# Autodesk Inventor assembly: Assembly
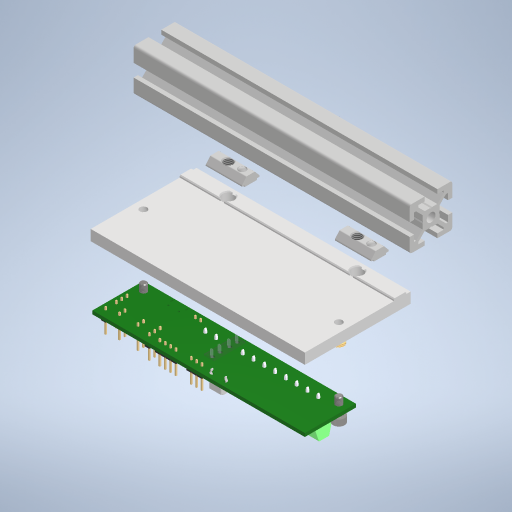
[picture p0: Inventor's stored thumbnail of the model, 512x512]
Saved by Autodesk Inventor 2023.1 (Build 271208000, 208)
## iProperties
Created: 2022-09-11
Part Number: Assembly
Document SubType Name: Assembly
Designer: Rama
Author: Rama
## Documents named in this file (8)
- C:\Users\Rama\Desktop\Mix\Klipper_Expander\CAD\Source\Assembly.iam
- C:\Users\Rama\Desktop\Mix\Klipper_Expander\CAD\Source\Klipper_Expander_Mount.ipt
- C:\Users\Rama\Documents\Inventor\Content Center Files\R2023\de-DE\ISO 7380-1\ISO 7380-1 - M5 x 8.ipt
- C:\Users\Rama\Desktop\GitHub\TrashInventor\HFSB5-2020-130.ipt
- C:\Users\Rama\Documents\Inventor\Content Center Files\R2023\de-DE\DIN 912\DIN 912 - M3 x 0,5 x 8 x 6,75.ipt
- C:\Users\Rama\Desktop\GitHub\TrashInventor\M3 Threaded Insert.ipt
- C:\Users\Rama\Desktop\GitHub\TrashInventor\SHNTP5-5.ipt
- C:\Users\Rama\Desktop\KE\STM32_Klipper_Expander.iam
## Components (11 placed, 7 different names)
1. Klipper_Expander_Mount:1 — Passend:1, Passend:2, Passend:7, Passend:8, Fluchtend:6
2. ISO 7380-1 M5 x 8:1 — Passend:1, Fluchtend:1, Passend:9
3. ISO 7380-1 M5 x 8:2 — Passend:2, Fluchtend:1, Passend:10
4. HFSB5-2020-130:1 — Passend:11, Winkel:1, Fluchtend:6
5. DIN 912 - ersetzt durch DIN EN ISO 4762 M3 x 8:1 — Fluchtend:2
6. DIN 912 - ersetzt durch DIN EN ISO 4762 M3 x 8:2 — Fluchtend:2
7. M3 Threaded Insert:1 — Passend:7, Fluchtend:3, Passend:12
8. M3 Threaded Insert:2 — Passend:8, Fluchtend:3, Passend:13
9. SHNTP5-5:1 — Passend:9, Fluchtend:4, Fluchtend:5, Passend:11, Winkel:1
10. SHNTP5-5:2 — Passend:10, Fluchtend:4, Fluchtend:5
11. STM32_Klipper_Expander:1 [sub-assembly] — Passend:12, Passend:13
## Relationships (16: Mate 9, Flush 6, Angle 1)
- Passend:1 [Mate]: Klipper_Expander_Mount:1 ↔ ISO 7380-1 M5 x 8:1
- Passend:2 [Mate]: Klipper_Expander_Mount:1 ↔ ISO 7380-1 M5 x 8:2
- Fluchtend:1 [Flush]: ISO 7380-1 M5 x 8:1 ↔ ISO 7380-1 M5 x 8:2
- Fluchtend:2 [Flush]: DIN 912 - ersetzt durch DIN EN ISO 4762 M3 x 8:1 ↔ DIN 912 - ersetzt durch DIN EN ISO 4762 M3 x 8:2
- Passend:7 [Mate]: Klipper_Expander_Mount:1 ↔ M3 Threaded Insert:1
- Passend:8 [Mate]: Klipper_Expander_Mount:1 ↔ M3 Threaded Insert:2
- Fluchtend:3 [Flush]: M3 Threaded Insert:1 ↔ M3 Threaded Insert:2
- Passend:9 [Mate]: ISO 7380-1 M5 x 8:1 ↔ SHNTP5-5:1
- Passend:10 [Mate]: ISO 7380-1 M5 x 8:2 ↔ SHNTP5-5:2
- Fluchtend:4 [Flush]: SHNTP5-5:1 ↔ SHNTP5-5:2
- Fluchtend:5 [Flush]: SHNTP5-5:1 ↔ SHNTP5-5:2
- Passend:11 [Mate] (0.1 mm): HFSB5-2020-130:1 ↔ SHNTP5-5:1
- Winkel:1 [Angle] (0 deg): HFSB5-2020-130:1 ↔ SHNTP5-5:1
- Fluchtend:6 [Flush] (-14.6 mm): Klipper_Expander_Mount:1 ↔ HFSB5-2020-130:1
- Passend:12 [Mate]: M3 Threaded Insert:1 ↔ STM32_Klipper_Expander:1
- Passend:13 [Mate]: M3 Threaded Insert:2 ↔ STM32_Klipper_Expander:1
